# Autodesk Inventor assembly: baseRoulante
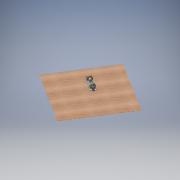
[picture p0: Inventor's stored thumbnail of the model, 180x180]
Saved by Autodesk Inventor 2017 (Build 210142000, 142)
## iProperties
Created: 2017-12-17
Part Number: baseRoulante
Document SubType Name: Assembly
Designer: franc
Author: franc
## Documents named in this file (10)
- C:\Users\franc\Desktop\EsialRobotik\Mecanique\base_roulante\baseRoulante.iam
- C:\Users\franc\Desktop\EsialRobotik\Mecanique\base_roulante\socle_ammovible.ipt
- C:\Users\franc\Desktop\EsialRobotik\Mecanique\base_roulante\bloc_moteur.iam
- C:\Users\franc\Desktop\EsialRobotik\Mecanique\base_roulante\composants\capuchon_roulement.ipt
- C:\Users\franc\Desktop\EsialRobotik\Mecanique\base_roulante\composants\LM4UU.ipt
- C:\Users\franc\Desktop\EsialRobotik\Mecanique\base_roulante\bloc_codeur.iam
- C:\Users\franc\Desktop\EsialRobotik\Mecanique\base_roulante\sol.ipt
- C:\Users\franc\Desktop\EsialRobotik\Mecanique\Content Center Files\R2017\fr-FR\BS 4183(5)\BS 4183 - M2 x 20(2) I.ipt
- C:\Users\franc\Desktop\EsialRobotik\Mecanique\base_roulante\axe_codeur.iam
- C:\Users\franc\Desktop\EsialRobotik\Mecanique\Content Center Files\R2017\fr-FR\CNS 4355\CNS 4355 - M 3 x 10.ipt
## Components (50 placed, 9 different names)
1. socle_ammovible:1 — Affleurement:4, Placage:18, Placage:19, Placage:20, Placage:21, Placage:22, Placage:23, Placage:29, Placage:30, Placage:32, Affleurement:5, Affleurement:6, Placage:35, Placage:36, Placage:41, Placage:42, Placage:43, Placage:49, Placage:50, Placage:51, Placage:52, Placage:60, Placage:61, Placage:62, Placage:63, Placage:64, Placage:65, Placage:70, Placage:71, Placage:72, Placage:73, Placage:78, Placage:79, Placage:80, Placage:81, Placage:82, Placage:83, Placage:92, Placage:93, Placage:94, Placage:95, Placage:100, Placage:101, Placage:102, Placage:103, Placage:104, Placage:105, Placage:106, Placage:107, Placage:108, Placage:109, Placage:110, Placage:111, Placage:112, Placage:113, Placage:114, Placage:115, Placage:116, Placage:117, Placage:118, Placage:119
2. bloc_moteur:1 [sub-assembly] — Placage:18, Placage:19, Placage:20, Tangente:1, Placage:88, Placage:89, Placage:90, Placage:91
3. bloc_moteur:2 [sub-assembly] — Placage:21, Placage:22, Placage:23, Placage:96, Placage:97, Placage:98, Placage:99
4. sol:1 — Tangente:1, Affleurement:5, Affleurement:6, Tangente:2, Tangente:3
5. CNS 4355 M 3 x 10:1 — Placage:91, Placage:95
6. CNS 4355 M 3 x 10:2 — Placage:90, Placage:94
7. CNS 4355 M 3 x 10:3 — Placage:89, Placage:93
8. CNS 4355 M 3 x 10:4 — Placage:88, Placage:92
9. CNS 4355 M 3 x 10:5 — Placage:98, Placage:102
10. CNS 4355 M 3 x 10:6 — Placage:97, Placage:101
11. CNS 4355 M 3 x 10:7 — Placage:96, Placage:100
12. CNS 4355 M 3 x 10:8 — Placage:99, Placage:103
13. CNS 4355 M 3 x 10:9 — Placage:107, Placage:108
14. CNS 4355 M 3 x 10:10 — Placage:106, Placage:109
15. CNS 4355 M 3 x 10:11 — Placage:105, Placage:110
16. CNS 4355 M 3 x 10:12 — Placage:104, Placage:111
17. CNS 4355 M 3 x 10:13 — Placage:112, Placage:119
18. CNS 4355 M 3 x 10:14 — Placage:113, Placage:118
19. CNS 4355 M 3 x 10:15 — Placage:114, Placage:117
20. CNS 4355 M 3 x 10:16 — Placage:115, Placage:116
21. BS 4183 Vis à tête cylindrique fendue - Métrique M2 x 20:10 — Placage:67, Placage:73
22. BS 4183 Vis à tête cylindrique fendue - Métrique M2 x 20:11 — Placage:66, Placage:72
23. BS 4183 Vis à tête cylindrique fendue - Métrique M2 x 20:12 — Placage:69, Placage:70
24. BS 4183 Vis à tête cylindrique fendue - Métrique M2 x 20:13 — Placage:68, Placage:71
25. BS 4183 Vis à tête cylindrique fendue - Métrique M2 x 20:14 — Placage:77, Placage:78
26. BS 4183 Vis à tête cylindrique fendue - Métrique M2 x 20:15 — Placage:76, Placage:80
27. BS 4183 Vis à tête cylindrique fendue - Métrique M2 x 20:16 — Placage:75, Placage:79
28. BS 4183 Vis à tête cylindrique fendue - Métrique M2 x 20:17 — Placage:74, Placage:81
29. BS 4183 Vis à tête cylindrique fendue - Métrique M2 x 20:1 — Placage:39, Placage:42
30. BS 4183 Vis à tête cylindrique fendue - Métrique M2 x 20:2 — Placage:37, Placage:43
31. BS 4183 Vis à tête cylindrique fendue - Métrique M2 x 20:3 — Placage:35, Placage:36
32. BS 4183 Vis à tête cylindrique fendue - Métrique M2 x 20:4 — Placage:38, Placage:41
33. BS 4183 Vis à tête cylindrique fendue - Métrique M2 x 20:5 — Placage:46, Placage:50
34. BS 4183 Vis à tête cylindrique fendue - Métrique M2 x 20:7 — Placage:47, Placage:52
35. BS 4183 Vis à tête cylindrique fendue - Métrique M2 x 20:8 — Placage:48, Placage:51
36. BS 4183 Vis à tête cylindrique fendue - Métrique M2 x 20:9 — Placage:45, Placage:49
37. axe_codeur:1 [sub-assembly] — Affleurement:11, Placage:120
38. axe_codeur:2 [sub-assembly] — Affleurement:10, Placage:121
39. capuchon_roulement:1 — Placage:24, Placage:25, Placage:29, Placage:34, Affleurement:7, Placage:37, Placage:38, Placage:39
40. capuchon_roulement:2 — Placage:27, Placage:28, Placage:30, Affleurement:8, Placage:44, Placage:45, Placage:46, Placage:47, Placage:48
41. LM4UU:3 — Placage:24, Placage:25, Placage:120
42. LM4UU:4 — Placage:27, Placage:28, Placage:121
43. bloc_codeur:1 [sub-assembly] — Placage:31, Placage:32, Placage:34, Affleurement:7, Affleurement:8, Placage:44, Affleurement:10, Affleurement:11, Tangente:2
44. capuchon_roulement:3 — Placage:56, Placage:58, Placage:63, Placage:64, Placage:65, Placage:66, Placage:67, Placage:68, Placage:69
45. capuchon_roulement:4 — Placage:57, Placage:59, Placage:60, Placage:61, Placage:62, Placage:74, Placage:75, Placage:76, Placage:77
46. LM4UU:5 — Placage:56, Placage:58, Placage:123
47. LM4UU:6 — Placage:57, Placage:59
48. axe_codeur:3 [sub-assembly] — Placage:82, Affleurement:12, Placage:123, Placage:124
49. axe_codeur:4 [sub-assembly] — Placage:83, Affleurement:13, Placage:125
50. bloc_codeur:2 [sub-assembly] — Affleurement:12, Affleurement:13, Placage:124, Placage:125, Tangente:3
## Relationships (109: Mate 97, Flush 9, Tangent 3)
- Affleurement:4 [Flush] (-46 mm): socle_ammovible:1
- Placage:18 [Mate]: socle_ammovible:1 ↔ bloc_moteur:1
- Placage:19 [Mate]: socle_ammovible:1 ↔ bloc_moteur:1
- Placage:20 [Mate]: socle_ammovible:1 ↔ bloc_moteur:1
- Placage:21 [Mate]: socle_ammovible:1 ↔ bloc_moteur:2
- Placage:22 [Mate]: socle_ammovible:1 ↔ bloc_moteur:2
- Placage:23 [Mate]: socle_ammovible:1 ↔ bloc_moteur:2
- Placage:24 [Mate]: capuchon_roulement:1 ↔ LM4UU:3
- Placage:25 [Mate]: capuchon_roulement:1 ↔ LM4UU:3
- Placage:27 [Mate]: capuchon_roulement:2 ↔ LM4UU:4
- Placage:28 [Mate]: capuchon_roulement:2 ↔ LM4UU:4
- Placage:29 [Mate]: socle_ammovible:1 ↔ capuchon_roulement:1
- Placage:30 [Mate]: socle_ammovible:1 ↔ capuchon_roulement:2
- Placage:31 [Mate]: bloc_codeur:1
- Placage:32 [Mate] (1 mm): socle_ammovible:1 ↔ bloc_codeur:1
- Tangente:1: bloc_moteur:1 ↔ sol:1
- Affleurement:5 [Flush] (500 mm): socle_ammovible:1 ↔ sol:1
- Affleurement:6 [Flush] (500 mm): socle_ammovible:1 ↔ sol:1
- Placage:34 [Mate] (3 mm): capuchon_roulement:1 ↔ bloc_codeur:1
- Affleurement:7 [Flush]: capuchon_roulement:1 ↔ bloc_codeur:1
- Placage:35 [Mate]: socle_ammovible:1 ↔ BS 4183 Vis à tête cylindrique fendue - Métrique M2 x 20:3
- Placage:36 [Mate]: socle_ammovible:1 ↔ BS 4183 Vis à tête cylindrique fendue - Métrique M2 x 20:3
- Placage:37 [Mate]: BS 4183 Vis à tête cylindrique fendue - Métrique M2 x 20:2 ↔ capuchon_roulement:1
- Placage:38 [Mate]: BS 4183 Vis à tête cylindrique fendue - Métrique M2 x 20:4 ↔ capuchon_roulement:1
- Placage:39 [Mate]: BS 4183 Vis à tête cylindrique fendue - Métrique M2 x 20:1 ↔ capuchon_roulement:1
- Placage:41 [Mate]: socle_ammovible:1 ↔ BS 4183 Vis à tête cylindrique fendue - Métrique M2 x 20:4
- Placage:42 [Mate]: socle_ammovible:1 ↔ BS 4183 Vis à tête cylindrique fendue - Métrique M2 x 20:1
- Placage:43 [Mate]: socle_ammovible:1 ↔ BS 4183 Vis à tête cylindrique fendue - Métrique M2 x 20:2
- Affleurement:8 [Flush]: capuchon_roulement:2 ↔ bloc_codeur:1
- Placage:44 [Mate] (3 mm): capuchon_roulement:2 ↔ bloc_codeur:1
- Placage:45 [Mate]: BS 4183 Vis à tête cylindrique fendue - Métrique M2 x 20:9 ↔ capuchon_roulement:2
- Placage:46 [Mate]: BS 4183 Vis à tête cylindrique fendue - Métrique M2 x 20:5 ↔ capuchon_roulement:2
- Placage:47 [Mate]: BS 4183 Vis à tête cylindrique fendue - Métrique M2 x 20:7 ↔ capuchon_roulement:2
- Placage:48 [Mate]: BS 4183 Vis à tête cylindrique fendue - Métrique M2 x 20:8 ↔ capuchon_roulement:2
- Placage:49 [Mate]: socle_ammovible:1 ↔ BS 4183 Vis à tête cylindrique fendue - Métrique M2 x 20:9
- Placage:50 [Mate]: socle_ammovible:1 ↔ BS 4183 Vis à tête cylindrique fendue - Métrique M2 x 20:5
- Placage:51 [Mate]: socle_ammovible:1 ↔ BS 4183 Vis à tête cylindrique fendue - Métrique M2 x 20:8
- Placage:52 [Mate]: socle_ammovible:1 ↔ BS 4183 Vis à tête cylindrique fendue - Métrique M2 x 20:7
- Affleurement:10 [Flush]: axe_codeur:2 ↔ bloc_codeur:1
- Affleurement:11 [Flush]: axe_codeur:1 ↔ bloc_codeur:1
- Placage:56 [Mate]: capuchon_roulement:3 ↔ LM4UU:5
- Placage:57 [Mate]: capuchon_roulement:4 ↔ LM4UU:6
- Placage:58 [Mate]: capuchon_roulement:3 ↔ LM4UU:5
- Placage:59 [Mate]: capuchon_roulement:4 ↔ LM4UU:6
- Placage:60 [Mate]: socle_ammovible:1 ↔ capuchon_roulement:4
- Placage:61 [Mate]: socle_ammovible:1 ↔ capuchon_roulement:4
- Placage:62 [Mate]: socle_ammovible:1 ↔ capuchon_roulement:4
- Placage:63 [Mate]: socle_ammovible:1 ↔ capuchon_roulement:3
- Placage:64 [Mate]: socle_ammovible:1 ↔ capuchon_roulement:3
- Placage:65 [Mate]: socle_ammovible:1 ↔ capuchon_roulement:3
- Placage:66 [Mate]: BS 4183 Vis à tête cylindrique fendue - Métrique M2 x 20:11 ↔ capuchon_roulement:3
- Placage:67 [Mate]: BS 4183 Vis à tête cylindrique fendue - Métrique M2 x 20:10 ↔ capuchon_roulement:3
- Placage:68 [Mate]: BS 4183 Vis à tête cylindrique fendue - Métrique M2 x 20:13 ↔ capuchon_roulement:3
- Placage:69 [Mate]: BS 4183 Vis à tête cylindrique fendue - Métrique M2 x 20:12 ↔ capuchon_roulement:3
- Placage:70 [Mate]: socle_ammovible:1 ↔ BS 4183 Vis à tête cylindrique fendue - Métrique M2 x 20:12
- Placage:71 [Mate]: socle_ammovible:1 ↔ BS 4183 Vis à tête cylindrique fendue - Métrique M2 x 20:13
- Placage:72 [Mate]: socle_ammovible:1 ↔ BS 4183 Vis à tête cylindrique fendue - Métrique M2 x 20:11
- Placage:73 [Mate]: socle_ammovible:1 ↔ BS 4183 Vis à tête cylindrique fendue - Métrique M2 x 20:10
- Placage:74 [Mate]: BS 4183 Vis à tête cylindrique fendue - Métrique M2 x 20:17 ↔ capuchon_roulement:4
- Placage:75 [Mate]: BS 4183 Vis à tête cylindrique fendue - Métrique M2 x 20:16 ↔ capuchon_roulement:4
- Placage:76 [Mate]: BS 4183 Vis à tête cylindrique fendue - Métrique M2 x 20:15 ↔ capuchon_roulement:4
- Placage:77 [Mate]: BS 4183 Vis à tête cylindrique fendue - Métrique M2 x 20:14 ↔ capuchon_roulement:4
- Placage:78 [Mate]: socle_ammovible:1 ↔ BS 4183 Vis à tête cylindrique fendue - Métrique M2 x 20:14
- Placage:79 [Mate]: socle_ammovible:1 ↔ BS 4183 Vis à tête cylindrique fendue - Métrique M2 x 20:16
- Placage:80 [Mate]: socle_ammovible:1 ↔ BS 4183 Vis à tête cylindrique fendue - Métrique M2 x 20:15
- Placage:81 [Mate]: socle_ammovible:1 ↔ BS 4183 Vis à tête cylindrique fendue - Métrique M2 x 20:17
- Placage:82 [Mate]: socle_ammovible:1 ↔ axe_codeur:3
- Placage:83 [Mate]: socle_ammovible:1 ↔ axe_codeur:4
- Affleurement:12 [Flush]: axe_codeur:3 ↔ bloc_codeur:2
- Placage:88 [Mate]: bloc_moteur:1 ↔ CNS 4355 M 3 x 10:4
- Placage:89 [Mate]: bloc_moteur:1 ↔ CNS 4355 M 3 x 10:3
- Placage:90 [Mate]: bloc_moteur:1 ↔ CNS 4355 M 3 x 10:2
- Placage:91 [Mate]: bloc_moteur:1 ↔ CNS 4355 M 3 x 10:1
- Placage:92 [Mate]: socle_ammovible:1 ↔ CNS 4355 M 3 x 10:4
- Placage:93 [Mate]: socle_ammovible:1 ↔ CNS 4355 M 3 x 10:3
- Placage:94 [Mate]: socle_ammovible:1 ↔ CNS 4355 M 3 x 10:2
- Placage:95 [Mate]: socle_ammovible:1 ↔ CNS 4355 M 3 x 10:1
- Placage:96 [Mate]: bloc_moteur:2 ↔ CNS 4355 M 3 x 10:7
- Placage:97 [Mate]: bloc_moteur:2 ↔ CNS 4355 M 3 x 10:6
- Placage:98 [Mate]: bloc_moteur:2 ↔ CNS 4355 M 3 x 10:5
- Placage:99 [Mate]: bloc_moteur:2 ↔ CNS 4355 M 3 x 10:8
- Placage:100 [Mate]: socle_ammovible:1 ↔ CNS 4355 M 3 x 10:7
- Placage:101 [Mate]: socle_ammovible:1 ↔ CNS 4355 M 3 x 10:6
- Placage:102 [Mate]: socle_ammovible:1 ↔ CNS 4355 M 3 x 10:5
- Placage:103 [Mate]: socle_ammovible:1 ↔ CNS 4355 M 3 x 10:8
- Placage:104 [Mate]: socle_ammovible:1 ↔ CNS 4355 M 3 x 10:12
- Placage:105 [Mate]: socle_ammovible:1 ↔ CNS 4355 M 3 x 10:11
- Placage:106 [Mate]: socle_ammovible:1 ↔ CNS 4355 M 3 x 10:10
- Placage:107 [Mate]: socle_ammovible:1 ↔ CNS 4355 M 3 x 10:9
- Placage:108 [Mate]: socle_ammovible:1 ↔ CNS 4355 M 3 x 10:9
- Placage:109 [Mate]: socle_ammovible:1 ↔ CNS 4355 M 3 x 10:10
- Placage:110 [Mate]: socle_ammovible:1 ↔ CNS 4355 M 3 x 10:11
- Placage:111 [Mate]: socle_ammovible:1 ↔ CNS 4355 M 3 x 10:12
- Placage:112 [Mate]: socle_ammovible:1 ↔ CNS 4355 M 3 x 10:13
- Placage:113 [Mate]: socle_ammovible:1 ↔ CNS 4355 M 3 x 10:14
- Placage:114 [Mate]: socle_ammovible:1 ↔ CNS 4355 M 3 x 10:15
- Placage:115 [Mate]: socle_ammovible:1 ↔ CNS 4355 M 3 x 10:16
- Placage:116 [Mate]: socle_ammovible:1 ↔ CNS 4355 M 3 x 10:16
- Placage:117 [Mate]: socle_ammovible:1 ↔ CNS 4355 M 3 x 10:15
- Placage:118 [Mate]: socle_ammovible:1 ↔ CNS 4355 M 3 x 10:14
- Placage:119 [Mate]: socle_ammovible:1 ↔ CNS 4355 M 3 x 10:13
- Placage:120 [Mate]: axe_codeur:1 ↔ LM4UU:3
- Placage:121 [Mate]: axe_codeur:2 ↔ LM4UU:4
- Placage:123 [Mate]: LM4UU:5 ↔ axe_codeur:3
- Affleurement:13 [Flush]: axe_codeur:4 ↔ bloc_codeur:2
- Placage:124 [Mate]: axe_codeur:3 ↔ bloc_codeur:2
- Placage:125 [Mate]: axe_codeur:4 ↔ bloc_codeur:2
- Tangente:2: sol:1 ↔ bloc_codeur:1
- Tangente:3: sol:1 ↔ bloc_codeur:2
